# Autodesk Inventor assembly: BrachV2
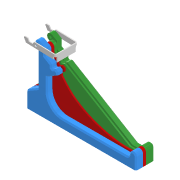
[picture p0: Inventor's stored thumbnail of the model, 180x180]
Saved by Autodesk Inventor 2020 (Build 240168000, 168)
## iProperties
Created: 2021-07-08
Part Number: BrachV2
Document SubType Name: Assembly
Designer: Aidan Lee
Author: Aidan Lee
## Documents named in this file (9)
- C:\Users\hobly\Dropbox\Aidan Lee\Mechanics_Walk\Brachistochrone-v2\BrachistochroneCurvedPaths.iam
- C:\Users\hobly\Dropbox\Aidan Lee\Mechanics_Walk\Brachistochrone-v2\BR-01-linerail.ipt
- C:\Users\hobly\Dropbox\Aidan Lee\Mechanics_Walk\Brachistochrone-v2\BR-03-cycloidrail.ipt
- C:\Users\hobly\Dropbox\Aidan Lee\Mechanics_Walk\Brachistochrone-v2\BR-04-cycloidpath.ipt
- C:\Users\hobly\Dropbox\Aidan Lee\Mechanics_Walk\Brachistochrone-v2\BR-02-linepath.ipt
- C:\Users\hobly\Dropbox\Aidan Lee\Mechanics_Walk\Brachistochrone-v2\BR-05-steeppath.ipt
- C:\Users\hobly\Dropbox\Aidan Lee\Mechanics_Walk\Brachistochrone-v2\BR-08-starter.ipt
- C:\Users\hobly\Dropbox\Aidan Lee\Mechanics_Walk\Brachistochrone-v2\BR-06-backrailline.ipt
- C:\Users\hobly\Dropbox\Aidan Lee\Mechanics_Walk\Brachistochrone-v2\BR-07-frontrailsteep.ipt
## Components (8 placed, 8 different names)
1. BR-01-linerail:1 — Mate:9, Flush:7, Flush:8, Mate:10, Flush:10
2. BR-03-cycloidrail:1 — Mate:7, Mate:8, Flush:6, Flush:8, Mate:19, Mate:20, Flush:13
3. BR-04-cycloidpath:1 — Mate:8, Flush:6, Mate:9, Flush:7, Flush:12
4. BR-02-linepath:1 — Mate:10, Flush:10, Mate:21, Flush:14
5. BR-05-steeppath:1 — Mate:7, Mate:17, Mate:18, Flush:11, Mate:19, Flush:12, Mate:20, Flush:13
6. BR-08-starter:1 — Mate:14, Mate:15
7. BR-06-backrailline:1 — Mate:21, Flush:14
8. BR-07-frontrailsteep:1 — Mate:11, Mate:12, Mate:13, Mate:14, Mate:15, Mate:17, Mate:18, Flush:11
## Relationships (22: Mate 14, Flush 8)
- Mate:7: BR-03-cycloidrail:1 ↔ BR-05-steeppath:1
- Mate:8: BR-03-cycloidrail:1 ↔ BR-04-cycloidpath:1
- Flush:6: BR-03-cycloidrail:1 ↔ BR-04-cycloidpath:1
- Mate:9: BR-01-linerail:1 ↔ BR-04-cycloidpath:1
- Flush:7: BR-01-linerail:1 ↔ BR-04-cycloidpath:1
- Flush:8: BR-01-linerail:1 ↔ BR-03-cycloidrail:1
- Mate:10: BR-01-linerail:1 ↔ BR-02-linepath:1
- Flush:10: BR-01-linerail:1 ↔ BR-02-linepath:1
- Mate:11: BR-07-frontrailsteep:1
- Mate:12: BR-07-frontrailsteep:1
- Mate:13: BR-07-frontrailsteep:1
- Mate:14: BR-08-starter:1 ↔ BR-07-frontrailsteep:1
- Mate:15 (2 mm): BR-08-starter:1 ↔ BR-07-frontrailsteep:1
- Mate:17: BR-05-steeppath:1 ↔ BR-07-frontrailsteep:1
- Mate:18: BR-05-steeppath:1 ↔ BR-07-frontrailsteep:1
- Flush:11: BR-05-steeppath:1 ↔ BR-07-frontrailsteep:1
- Mate:19: BR-03-cycloidrail:1 ↔ BR-05-steeppath:1
- Flush:12: BR-04-cycloidpath:1 ↔ BR-05-steeppath:1
- Mate:20: BR-03-cycloidrail:1 ↔ BR-05-steeppath:1
- Flush:13: BR-03-cycloidrail:1 ↔ BR-05-steeppath:1
- Mate:21: BR-02-linepath:1 ↔ BR-06-backrailline:1
- Flush:14: BR-02-linepath:1 ↔ BR-06-backrailline:1
